# Autodesk Inventor assembly: Laboratorio
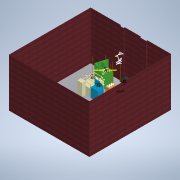
[picture p0: Inventor's stored thumbnail of the model, 180x180]
Saved by Autodesk Inventor 2020 (Build 240168000, 168)
## iProperties
Created: 2019-10-05
Part Number: Laboratorio
Document SubType Name: Assembly
Designer: dasa1
Author: dasa1
## Documents named in this file (9)
- C:\Users\dasa1\OneDrive\Documents\Inventor\Virtualización Maya\Laboratorio.iam
- C:\Users\dasa1\OneDrive\Documents\Inventor\Virtualización Maya\Entorno.ipt
- C:\Users\dasa1\OneDrive\Documents\Inventor\Virtualización Maya\multiejes.ipt
- C:\Users\dasa1\OneDrive\Documents\Inventor\Virtualización Maya\Gantry.ipt
- C:\Users\dasa1\OneDrive\Documents\Inventor\Virtualización Maya\Mesa piezas.ipt
- C:\Users\dasa1\OneDrive\Documents\Inventor\Virtualización Maya\Tablero Maya.ipt
- C:\Users\dasa1\OneDrive\Documents\Inventor\Virtualización Maya\Tablero Eléctrico.ipt
- C:\Users\dasa1\OneDrive\Documents\Inventor\Virtualización Maya\CMM.ipt
- C:\Users\dasa1\OneDrive\Documents\Inventor\Virtualización Maya\SDV.ipt
## Components (8 placed, 8 different names)
1. Entorno:1 — Coincidencia:4, Coincidencia:5, Coincidencia:6, Coincidencia:7, Coincidencia:9, Coincidencia:10, Coincidencia:12, Coincidencia:13, Coincidencia:15, Coincidencia:18, Coincidencia:20, Ángulo:2, Coincidencia:22, Coincidencia:23, Ángulo:3, Coincidencia:24, Ángulo:4, Coincidencia:26, Coincidencia:28, Coincidencia:29, Ángulo:7, Ángulo:8, Coincidencia:30, Coincidencia:31
2. multiejes:1 — Coincidencia:26, Coincidencia:27, Ángulo:6, Ángulo:8
3. Mesa piezas:1 — Coincidencia:7, Coincidencia:9, Coincidencia:22, Ángulo:9
4. Tablero Maya:1 — Coincidencia:10, Coincidencia:12, Coincidencia:29
5. Tablero Eléctrico:1 — Coincidencia:13, Coincidencia:15
6. CMM:1 — Coincidencia:18, Coincidencia:19, Ángulo:1, Ángulo:7
7. Gantry:1 — Coincidencia:4, Coincidencia:5, Coincidencia:6, Coincidencia:25, Ángulo:5
8. SDV:1 — Coincidencia:30, Coincidencia:31, Ángulo:9
## Relationships (32: Mate 23, Angle 9)
- Coincidencia:4 [Mate]: Entorno:1 ↔ Gantry:1
- Coincidencia:5 [Mate]: Entorno:1 ↔ Gantry:1
- Coincidencia:6 [Mate]: Entorno:1 ↔ Gantry:1
- Coincidencia:7 [Mate]: Entorno:1 ↔ Mesa piezas:1
- Coincidencia:9 [Mate]: Entorno:1 ↔ Mesa piezas:1
- Coincidencia:10 [Mate]: Entorno:1 ↔ Tablero Maya:1
- Coincidencia:12 [Mate] (370 mm): Entorno:1 ↔ Tablero Maya:1
- Coincidencia:13 [Mate]: Entorno:1 ↔ Tablero Eléctrico:1
- Coincidencia:15 [Mate] (2210 mm): Entorno:1 ↔ Tablero Eléctrico:1
- Coincidencia:18 [Mate]: Entorno:1 ↔ CMM:1
- Coincidencia:19 [Mate]: CMM:1
- Ángulo:1 [Angle] (0 deg): CMM:1
- Coincidencia:20 [Mate]: Entorno:1
- Ángulo:2 [Angle] (0 deg): Entorno:1
- Coincidencia:21 [Mate]
- Coincidencia:22 [Mate]: Entorno:1 ↔ Mesa piezas:1
- Coincidencia:23 [Mate]: Entorno:1
- Ángulo:3 [Angle] (0 deg): Entorno:1
- Coincidencia:24 [Mate]: Entorno:1
- Ángulo:4 [Angle] (0 deg): Entorno:1
- Coincidencia:25 [Mate]: Gantry:1
- Ángulo:5 [Angle] (0 deg): Gantry:1
- Coincidencia:26 [Mate]: Entorno:1 ↔ multiejes:1
- Coincidencia:27 [Mate]: multiejes:1
- Ángulo:6 [Angle] (0 deg): multiejes:1
- Coincidencia:28 [Mate]: Entorno:1
- Coincidencia:29 [Mate]: Entorno:1 ↔ Tablero Maya:1
- Ángulo:7 [Angle] (-90 deg): Entorno:1 ↔ CMM:1
- Ángulo:8 [Angle] (-95 deg): Entorno:1 ↔ multiejes:1
- Coincidencia:30 [Mate] (175 mm): Entorno:1 ↔ SDV:1
- Coincidencia:31 [Mate]: Entorno:1 ↔ SDV:1
- Ángulo:9 [Angle] (180 deg): Mesa piezas:1 ↔ SDV:1
